# Autodesk Inventor assembly: enc-FrontPanel Oben - Assembly no Absorber
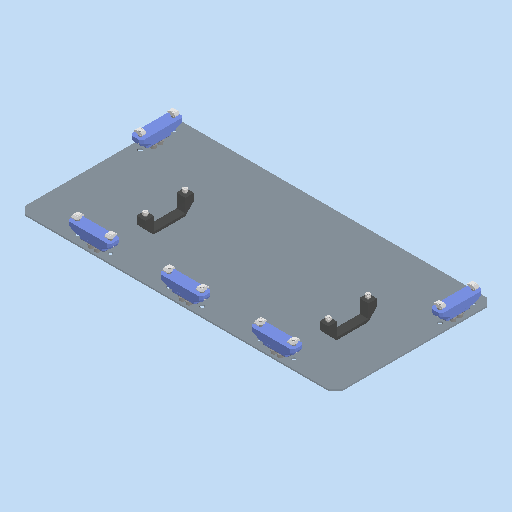
[picture p0: Inventor's stored thumbnail of the model, 512x512]
Saved by Autodesk Inventor 2023.2 (Build 272271000, 271)
## iProperties
Created: 2023-11-30
Part Number: enc-FrontPanel Oben - Assembly no Absorber
Document SubType Name: Assembly
Designer: Nils Bade
Author: Nils Bade
## Documents named in this file (6)
- C:\Users\nilsb\Documents\Inventor\Projektarbeit-Bade\Enclosure\enc-FrontPanel Oben - Assembly no Absorber.iam
- C:\Users\nilsb\Documents\Inventor\Projektarbeit-Bade\Enclosure\V-Slot Door Handle v1.ipt
- C:\Users\nilsb\Documents\Inventor\Projektarbeit-Bade\Schrauben\Cap Head Screw M6x16 - DIN912.ipt
- C:\Users\nilsb\Documents\Inventor\Projektarbeit-Bade\RatRig_Standards\Hex Locking Nut - M6 v2.ipt
- C:\Users\nilsb\Documents\Inventor\Projektarbeit-Bade\Enclosure\Magnet PanelFrame Straight connected.iam
- C:\Users\nilsb\Documents\Inventor\Projektarbeit-Bade\Enclosure\enc-FrontPanel Oben 357x708.ipt
## Components (16 placed, 5 different names)
1. enc-SidePanel Oben 357x708:2
2. V-Slot Door Handle v1:1 — Passend:11, Passend:12
3. V-Slot Door Handle v1:2 — Passend:9, Passend:10, Passend:13, Passend:14
4. Cap Head Screw M6x16 - DIN912:1 — Passend:12, Passend:17
5. Cap Head Screw M6x16 - DIN912:2 — Passend:11, Passend:18
6. Cap Head Screw M6x16 - DIN912:3 — Passend:9, Passend:13, Passend:15
7. Cap Head Screw M6x16 - DIN912:4 — Passend:10, Passend:14, Passend:16
8. Hex Locking Nut - M6 v2:1 — Passend:18
9. Hex Locking Nut - M6 v2:2 — Passend:17
10. Hex Locking Nut - M6 v2:3 — Passend:16
11. Hex Locking Nut - M6 v2:4 — Passend:15
12. Magnet PanelFrame Straight connected:1 [sub-assembly]
13. Magnet PanelFrame Straight connected:2 [sub-assembly]
14. Magnet PanelFrame Straight connected:3 [sub-assembly]
15. Magnet PanelFrame Straight connected:4 [sub-assembly]
16. Magnet PanelFrame Straight connected:5 [sub-assembly]
## Relationships (37: Mate 37)
- [Mate]: enc-SidePanel Oben 357x708:2 ↔ V-Slot Door Handle v1:1
- [Mate]: enc-SidePanel Oben 357x708:2 ↔ V-Slot Door Handle v1:1
- [Mate]: enc-SidePanel Oben 357x708:2 ↔ V-Slot Door Handle v1:1
- [Mate]: enc-SidePanel Oben 357x708:2 ↔ V-Slot Door Handle v1:2
- [Mate]: enc-SidePanel Oben 357x708:2 ↔ V-Slot Door Handle v1:2
- [Mate]: enc-SidePanel Oben 357x708:2 ↔ V-Slot Door Handle v1:2
- [Mate]: enc-SidePanel Oben 357x708:2 ↔ Cap Head Screw M6x16 - DIN912:1
- [Mate]: enc-SidePanel Oben 357x708:2 ↔ Cap Head Screw M6x16 - DIN912:2
- Passend:9 [Mate]: V-Slot Door Handle v1:2 ↔ Cap Head Screw M6x16 - DIN912:3
- Passend:10 [Mate]: V-Slot Door Handle v1:2 ↔ Cap Head Screw M6x16 - DIN912:4
- Passend:11 [Mate]: V-Slot Door Handle v1:1 ↔ Cap Head Screw M6x16 - DIN912:2
- Passend:12 [Mate]: V-Slot Door Handle v1:1 ↔ Cap Head Screw M6x16 - DIN912:1
- Passend:13 [Mate]: V-Slot Door Handle v1:2 ↔ Cap Head Screw M6x16 - DIN912:3
- Passend:14 [Mate]: V-Slot Door Handle v1:2 ↔ Cap Head Screw M6x16 - DIN912:4
- Passend:15 [Mate]: Cap Head Screw M6x16 - DIN912:3 ↔ Hex Locking Nut - M6 v2:4
- Passend:16 [Mate]: Cap Head Screw M6x16 - DIN912:4 ↔ Hex Locking Nut - M6 v2:3
- Passend:17 [Mate]: Cap Head Screw M6x16 - DIN912:1 ↔ Hex Locking Nut - M6 v2:2
- Passend:18 [Mate]: Cap Head Screw M6x16 - DIN912:2 ↔ Hex Locking Nut - M6 v2:1
- [Mate]: enc-SidePanel Oben 357x708:2 ↔ Hex Locking Nut - M6 v2:4
- [Mate]: enc-SidePanel Oben 357x708:2 ↔ Hex Locking Nut - M6 v2:3
- [Mate]: enc-SidePanel Oben 357x708:2 ↔ Hex Locking Nut - M6 v2:2
- [Mate]: enc-SidePanel Oben 357x708:2 ↔ Hex Locking Nut - M6 v2:1
- [Mate]: enc-SidePanel Oben 357x708:2 ↔ Magnet PanelFrame Straight connected:2
- [Mate]: enc-SidePanel Oben 357x708:2 ↔ Magnet PanelFrame Straight connected:2
- [Mate]: enc-SidePanel Oben 357x708:2 ↔ Magnet PanelFrame Straight connected:2
- [Mate]: enc-SidePanel Oben 357x708:2 ↔ Magnet PanelFrame Straight connected:1
- [Mate]: enc-SidePanel Oben 357x708:2 ↔ Magnet PanelFrame Straight connected:1
- [Mate]: enc-SidePanel Oben 357x708:2 ↔ Magnet PanelFrame Straight connected:1
- [Mate]: enc-SidePanel Oben 357x708:2 ↔ Magnet PanelFrame Straight connected:5
- [Mate]: enc-SidePanel Oben 357x708:2 ↔ Magnet PanelFrame Straight connected:5
- [Mate]: enc-SidePanel Oben 357x708:2 ↔ Magnet PanelFrame Straight connected:4
- [Mate]: enc-SidePanel Oben 357x708:2 ↔ Magnet PanelFrame Straight connected:4
- [Mate]: enc-SidePanel Oben 357x708:2 ↔ Magnet PanelFrame Straight connected:3
- [Mate]: enc-SidePanel Oben 357x708:2 ↔ Magnet PanelFrame Straight connected:3
- [Mate]: enc-SidePanel Oben 357x708:2 ↔ Magnet PanelFrame Straight connected:3
- [Mate]: enc-SidePanel Oben 357x708:2 ↔ Magnet PanelFrame Straight connected:4
- [Mate]: enc-SidePanel Oben 357x708:2 ↔ Magnet PanelFrame Straight connected:5
